# Autodesk Inventor assembly: Square_Cell
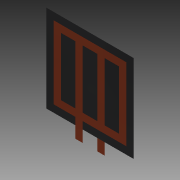
[picture p0: Inventor's stored thumbnail of the model, 180x180]
Saved by Autodesk Inventor 2014 SP1 (Build 180222100, 222)
## iProperties
Created: 2014-01-12
Part Number: Square_Cell
Document SubType Name: Assembly
Designer: tuleu
Author: tuleu
## Documents named in this file (3)
- C:\Users\tuleu\Documents\giant-snes-gamepad\cad\Square_Cell.iam
- C:\Users\tuleu\Documents\giant-snes-gamepad\cad\Square_Velostat.ipt
- C:\Users\tuleu\Documents\giant-snes-gamepad\cad\Square_Copper.ipt
## Components (3 placed, 2 different names)
1. Square_Velostat:1 — Flush:1, Mate:1, Flush:2, Mate:2, Mate:4, Mate:5, Mate:6
2. Square_Copper:1 — Flush:1, Mate:1, Flush:2
3. Square_Copper:2 — Mate:2, Mate:3, Mate:4
## Relationships (8: Mate 6, Flush 2)
- Flush:1: Square_Velostat:1 ↔ Square_Copper:1
- Mate:1: Square_Velostat:1 ↔ Square_Copper:1
- Flush:2: Square_Velostat:1 ↔ Square_Copper:1
- Mate:2: Square_Velostat:1 ↔ Square_Copper:2
- Mate:3: Square_Copper:2
- Mate:4: Square_Velostat:1 ↔ Square_Copper:2
- Mate:5: Square_Velostat:1
- Mate:6: Square_Velostat:1
